# Autodesk Inventor assembly: 10-1 Assembly
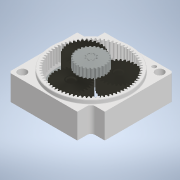
[picture p0: Inventor's stored thumbnail of the model, 180x180]
Saved by Autodesk Inventor 2020 (Build 240168000, 168)
## iProperties
Created: 2020-01-30
Part Number: 10-1 Assembly
Document SubType Name: Assembly
Designer: aidan
Author: aidan
## Documents named in this file (5)
- C:\Users\aidan\Desktop\T3 Robotics\CAD\Generic and Stock\10-1 Planetary Kit\10-1 Assembly.iam
- C:\Users\aidan\Desktop\T3 Robotics\CAD\Generic and Stock\10-1 Planetary Kit\VersaPlanetary 10-1 Base Gear.ipt
- C:\Users\aidan\Desktop\T3 Robotics\CAD\Generic and Stock\10-1 Planetary Kit\VersaPlanetary 10-1 Planet Gear.ipt
- C:\Users\aidan\Desktop\T3 Robotics\CAD\Generic and Stock\10-1 Planetary Kit\VersaPlanetary 10-1 Sun Gear.ipt
- C:\Users\aidan\Desktop\T3 Robotics\CAD\Generic and Stock\VersaPlanetary Ring Gear.ipt
## Components (6 placed, 4 different names)
1. VersaPlanetary 10-1 Base Gear:1 — Mate:1, Mate:2, Mate:3, Flush:1, Flush:2, Flush:3, Mate:5, Mate:8, Rotation:4
2. VersaPlanetary 10-1 Planet Gear:1 — Mate:2, Flush:1, Rotation:1, Rotation:2, Rotation:3, Flush:5, Tangent:1
3. VersaPlanetary 10-1 Planet Gear:2 — Mate:3, Flush:2, Mate:4, Rotation:1
4. VersaPlanetary 10-1 Planet Gear:3 — Mate:1, Flush:3, Rotation:2
5. VersaPlanetary 10-1 Sun Gear:1 — Mate:4, Mate:6, Rotation:3, Rotation:4
6. VersaPlanetary Ring Gear:1 — Flush:4, Mate:8, Flush:5, Tangent:1
## Relationships (18: Mate 8, Flush 5, RelateRotation 4, Tangent 1)
- Mate:1: VersaPlanetary 10-1 Base Gear:1 ↔ VersaPlanetary 10-1 Planet Gear:3
- Mate:2: VersaPlanetary 10-1 Base Gear:1 ↔ VersaPlanetary 10-1 Planet Gear:1
- Mate:3: VersaPlanetary 10-1 Base Gear:1 ↔ VersaPlanetary 10-1 Planet Gear:2
- Flush:1: VersaPlanetary 10-1 Base Gear:1 ↔ VersaPlanetary 10-1 Planet Gear:1
- Flush:2: VersaPlanetary 10-1 Base Gear:1 ↔ VersaPlanetary 10-1 Planet Gear:2
- Flush:3: VersaPlanetary 10-1 Base Gear:1 ↔ VersaPlanetary 10-1 Planet Gear:3
- Mate:4: VersaPlanetary 10-1 Planet Gear:2 ↔ VersaPlanetary 10-1 Sun Gear:1
- Mate:5: VersaPlanetary 10-1 Base Gear:1
- Mate:6: VersaPlanetary 10-1 Sun Gear:1
- Mate:7
- Rotation:1 [RelateRotation] (1 ul): VersaPlanetary 10-1 Planet Gear:1 ↔ VersaPlanetary 10-1 Planet Gear:2
- Rotation:2 [RelateRotation] (1 ul): VersaPlanetary 10-1 Planet Gear:1 ↔ VersaPlanetary 10-1 Planet Gear:3
- Rotation:3 [RelateRotation] (4 ul): VersaPlanetary 10-1 Planet Gear:1 ↔ VersaPlanetary 10-1 Sun Gear:1
- Flush:4: VersaPlanetary Ring Gear:1
- Mate:8: VersaPlanetary 10-1 Base Gear:1 ↔ VersaPlanetary Ring Gear:1
- Flush:5: VersaPlanetary 10-1 Planet Gear:1 ↔ VersaPlanetary Ring Gear:1
- Tangent:1: VersaPlanetary 10-1 Planet Gear:1 ↔ VersaPlanetary Ring Gear:1
- Rotation:4 [RelateRotation] (10 ul): VersaPlanetary 10-1 Base Gear:1 ↔ VersaPlanetary 10-1 Sun Gear:1
